# Autodesk Inventor assembly: ASY МОО 001 отстойник осветлитель
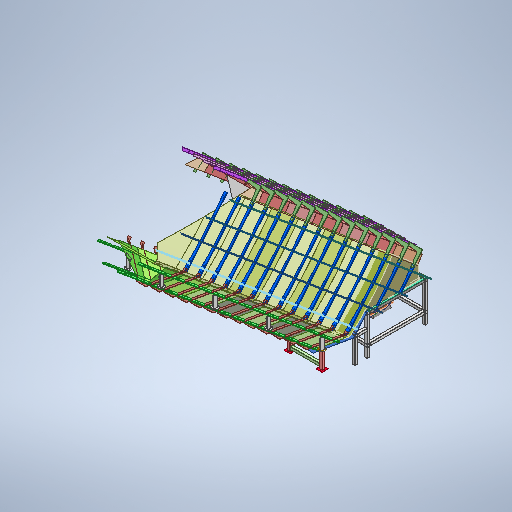
[picture p0: Inventor's stored thumbnail of the model, 512x512]
Saved by Autodesk Inventor 2025 (Build 290162010, 162A)
## iProperties
Created: 2024-04-28
Part Number: ASY МОО 001 отстойник осветлитель
Document SubType Name: Weldment
Designer: admin
Weld Material: Welded Aluminum-6061
Mass: 3.05393e+07 g
Surface Area: 3.06781e+06 cm^2
Volume: 2.84022e+07 cm^3
Density: 1.07525 g/cm^3
Author: admin
## Documents named in this file (61)
- C:\Users\admin\YandexDisk-badmisterfox\домашниий пк\Inventor\Manturovo\Manturovo_Se-clar\ASY МОО 001 отстойник осветлитель.iam
- C:\Users\admin\YandexDisk-badmisterfox\домашниий пк\Inventor\Manturovo\Manturovo_Se-clar\Пример емкости.ipt
- C:\Users\admin\YandexDisk-badmisterfox\домашниий пк\Inventor\Manturovo\Manturovo_Se-clar\Рама основания\ASY MSC 090 base frame.iam
- C:\Users\admin\YandexDisk-badmisterfox\домашниий пк\Inventor\Manturovo\Manturovo_Se-clar\ASY MSC 080 roсket.iam
- C:\Users\admin\YandexDisk-badmisterfox\домашниий пк\Inventor\Manturovo\Manturovo_Se-clar\ASY MSC 010 cone.iam
- C:\Users\admin\YandexDisk-badmisterfox\домашниий пк\Inventor\Manturovo\Manturovo_Se-clar\ракета\МОО 064 ракета труба.ipt
- C:\Users\admin\YandexDisk-badmisterfox\домашниий пк\Inventor\Manturovo\Manturovo_Se-clar\MSC 000 DIM settler-clarifier.ipt
- C:\Users\admin\YandexDisk-badmisterfox\домашниий пк\Inventor\Manturovo\Manturovo_Se-clar\MSC 031 sheet lowerback.ipt
- C:\Users\admin\YandexDisk-badmisterfox\домашниий пк\Inventor\Manturovo\Manturovo_Se-clar\MSC 021 sheet left board hip.ipt
- C:\Users\admin\YandexDisk-badmisterfox\домашниий пк\Inventor\Manturovo\Manturovo_Se-clar\MSC 022 sheet right board hip.ipt
- C:\Users\admin\YandexDisk-badmisterfox\домашниий пк\Inventor\Manturovo\Manturovo_Se-clar\конус\MSC 071 ridge 1.ipt
- C:\Users\admin\YandexDisk-badmisterfox\домашниий пк\Inventor\Manturovo\Manturovo_Se-clar\конус\MSC 073 ridge 3.ipt
- C:\Users\admin\YandexDisk-badmisterfox\домашниий пк\Inventor\Manturovo\Manturovo_Se-clar\конус\MSC 074 face 1.ipt
- C:\Users\admin\YandexDisk-badmisterfox\домашниий пк\Inventor\Manturovo\Manturovo_Se-clar\Content Center Files\en-US\ISO 5251 B 3D\ISO 5251 Bends 3D without straight ends(90 deg) DN150 11 11.ipt
- C:\Users\admin\YandexDisk-badmisterfox\домашниий пк\Inventor\Manturovo\Manturovo_Se-clar\Content Center Files\en-US\DIN EN 1092-1 01 - PN 25\DIN EN 1092-1 Plate Flange for Welding Type 01 - PN 25 150 x 168.3.ipt
- C:\Users\admin\YandexDisk-badmisterfox\домашниий пк\Inventor\Manturovo\Manturovo_Se-clar\МОО 061 труба верх 1.ipt
- C:\Users\admin\YandexDisk-badmisterfox\домашниий пк\Inventor\Manturovo\Manturovo_Se-clar\МОО 062 труба верх 2.ipt
- C:\Users\admin\YandexDisk-badmisterfox\домашниий пк\Inventor\Manturovo\Manturovo_Se-clar\МОО 063 труба верх 3.ipt
- C:\Users\admin\YandexDisk-badmisterfox\домашниий пк\Inventor\Manturovo\Manturovo_Se-clar\Part1.ipt
- C:\Users\admin\YandexDisk-badmisterfox\домашниий пк\Inventor\Manturovo\Manturovo_Se-clar\стапель\ASY стапель.iam
- C:\Users\admin\YandexDisk-badmisterfox\домашниий пк\Inventor\Manturovo\Manturovo_Se-clar\MSC 0101 sheet gills.ipt
- C:\Users\admin\YandexDisk-badmisterfox\домашниий пк\Inventor\Manturovo\Manturovo_Se-clar\MSC 068 stringer lowerback.ipt
- C:\Users\admin\YandexDisk-badmisterfox\домашниий пк\Inventor\Manturovo\Manturovo_Se-clar\конус\MSC 072 ridge 2.ipt
- C:\Users\admin\YandexDisk-badmisterfox\домашниий пк\Inventor\Manturovo\Manturovo_Se-clar\MSC 075 face 2.ipt
- C:\Users\admin\YandexDisk-badmisterfox\домашниий пк\Inventor\Manturovo\Manturovo_Se-clar\MSC 076 face 3.ipt
- C:\Users\admin\YandexDisk-badmisterfox\домашниий пк\Inventor\Manturovo\Manturovo_Se-clar\MSC 077 face 4.ipt
- C:\Users\admin\YandexDisk-badmisterfox\домашниий пк\Inventor\Manturovo\Manturovo_Se-clar\MSC 110 revision hatch 1.ipt
- C:\Users\admin\YandexDisk-badmisterfox\домашниий пк\Inventor\Manturovo\Manturovo_Se-clar\MSC 035 ring.ipt
- C:\Users\admin\YandexDisk-badmisterfox\домашниий пк\Inventor\Manturovo\Manturovo_Se-clar\MSC 074 ridge 4.ipt
- C:\Users\admin\YandexDisk-badmisterfox\домашниий пк\Inventor\Manturovo\Manturovo_Se-clar\MSC 075 ridge 5.ipt
- C:\Users\admin\YandexDisk-badmisterfox\домашниий пк\Inventor\Manturovo\Manturovo_Se-clar\MSC 081 pillar 1.ipt
- C:\Users\admin\YandexDisk-badmisterfox\домашниий пк\Inventor\Manturovo\Manturovo_Se-clar\MSC 036 flange 500.ipt
- C:\Users\admin\YandexDisk-badmisterfox\домашниий пк\Inventor\Manturovo\Manturovo_Se-clar\MSC 037 flange cover 500.ipt
- C:\Users\admin\YandexDisk-badmisterfox\домашниий пк\Inventor\Manturovo\Manturovo_Se-clar\MSC 038 flange cover ring 500.ipt
- C:\Users\admin\YandexDisk-badmisterfox\домашниий пк\Inventor\Manturovo\Manturovo_Se-clar\MSC 039 flange cover plate 500.ipt
- C:\Users\admin\YandexDisk-badmisterfox\домашниий пк\Inventor\Manturovo\Manturovo_Se-clar\Content Center Files\en-US\DIN EN ISO 8676\DIN EN ISO 8676 - M12 x 1,5 x 30.ipt
- C:\Users\admin\YandexDisk-badmisterfox\домашниий пк\Inventor\Manturovo\Manturovo_Se-clar\Content Center Files\en-US\ISO 4032(2)\ISO 4032 - M12 - ISO.ipt
- C:\Users\admin\YandexDisk-badmisterfox\домашниий пк\Inventor\Manturovo\Manturovo_Se-clar\Рама основания\ASY MSC 120  base frame.iam
- C:\Users\admin\YandexDisk-badmisterfox\домашниий пк\Inventor\Manturovo\Manturovo_Se-clar\Рама основания\ASY MSC 121  base frame.iam
- C:\Users\admin\YandexDisk-badmisterfox\домашниий пк\Inventor\Manturovo\Manturovo_Se-clar\Чертеж для парам. рамы.ipt
- C:\Users\admin\YandexDisk-badmisterfox\домашниий пк\Inventor\Manturovo\Manturovo_Se-clar\ASY MSC 120.1  base frame.iam
- C:\Users\admin\YandexDisk-badmisterfox\домашниий пк\Inventor\Manturovo\Manturovo_Se-clar\ASY MSC 122  base frame.iam
- C:\Users\admin\YandexDisk-badmisterfox\домашниий пк\Inventor\Manturovo\Manturovo_Se-clar\ASY MSC 123  base frame.iam
- C:\Users\admin\YandexDisk-badmisterfox\домашниий пк\Inventor\Manturovo\Manturovo_Se-clar\ASY MSC 124  base frame.iam
- C:\Users\admin\YandexDisk-badmisterfox\домашниий пк\Inventor\Manturovo\Manturovo_Se-clar\MSC 125 base tube.ipt
- C:\Users\admin\YandexDisk-badmisterfox\домашниий пк\Inventor\Manturovo\Manturovo_Se-clar\MSC 126 flange base tube.ipt
- C:\Users\admin\YandexDisk-badmisterfox\домашниий пк\Inventor\Manturovo\Manturovo_Se-clar\MSC 128 flange base tube support.ipt
- C:\Users\admin\YandexDisk-badmisterfox\домашниий пк\Inventor\Manturovo\Manturovo_Se-clar\MSC 125 base tube_MIR2.ipt
- C:\Users\admin\YandexDisk-badmisterfox\домашниий пк\Inventor\Manturovo\Manturovo_Se-clar\DXF файлы\MSC 126 flange base tube_MIR2.ipt
- C:\Users\admin\YandexDisk-badmisterfox\домашниий пк\Inventor\Manturovo\Manturovo_Se-clar\DXF файлы\MSC 128 flange base tube support_MIR1.ipt
- C:\Users\admin\YandexDisk-badmisterfox\домашниий пк\Inventor\Manturovo\Manturovo_Se-clar\ASY MSC 201 BACK.iam
- C:\Users\admin\YandexDisk-badmisterfox\домашниий пк\Inventor\Manturovo\Manturovo_Se-clar\ASY MSC 202 LEFT BOARD.iam
- C:\Users\admin\YandexDisk-badmisterfox\домашниий пк\Inventor\Manturovo\Manturovo_Se-clar\ASY MSC 203 RIGHT BOARD.iam
- C:\Users\admin\YandexDisk-badmisterfox\домашниий пк\Inventor\Manturovo\Manturovo_Se-clar\ASY MSC 204 BELLY.iam
- C:\Users\admin\YandexDisk-badmisterfox\домашниий пк\Inventor\Manturovo\Manturovo_Se-clar\MSC 063 stringer board #.ipt
- C:\Users\admin\YandexDisk-badmisterfox\домашниий пк\Inventor\Manturovo\Manturovo_Se-clar\MSC 064 stringer board ##.ipt
- C:\Users\admin\YandexDisk-badmisterfox\домашниий пк\Inventor\Manturovo\Manturovo_Se-clar\MSC 055 rib hip 2.ipt
- C:\Users\admin\YandexDisk-badmisterfox\домашниий пк\Inventor\Manturovo\Manturovo_Se-clar\MSC 054 rib hip 1.ipt
- C:\Users\admin\YandexDisk-badmisterfox\домашниий пк\Inventor\Manturovo\Manturovo_Se-clar\MSC 077 screen pillar .iam
- C:\Users\admin\YandexDisk-badmisterfox\домашниий пк\Inventor\Manturovo\Manturovo_Se-clar\MSC 0102 sheet gills.ipt
- C:\Users\admin\YandexDisk-badmisterfox\домашниий пк\Inventor\Manturovo\Manturovo_Se-clar\MSC 078 creen pillar.iam
## Components (131 placed, 62 different names)
1. Пример емкости.ipt:1 — Mate:1, Mate:2, Flush:2
2. MSC 000 DIM settler-clarifier.ipt:1
3. ASY MSC 090 base frame.iam:1 [sub-assembly] — Flush:19, Flush:21, Flush:82, Mate:82
4. ASY MSC 010 cone.iam:1 [sub-assembly] — Flush:22, Mate:16, Flush:28, Mate:65, Mate:78, Tangent:11, Flush:79, Mate:82, Mate:83
5. ASY MSC 080 roсket.iam:1 [sub-assembly] — Flush:23
6. МОО 064 ракета труба.ipt:1
7. MSC 031 sheet lowerback.ipt:1 — Mate:15, Mate:16, Tangent:10, Tangent:11, Tangent:12, Cylindrical:2, Rigid:185
8. MSC 021 sheet left board hip.ipt:1 — Flush:41, Mate:78
9. MSC 022 sheet right board hip.ipt:1 — Mate:30
10. MSC 071 ridge 1.ipt:1 — Mate:50, Flush:57, Mate:68, Flush:81, Flush:83, Mate:85
11. MSC 074 face 1.ipt:1 — Rigid:156, Rigid:157, Flush:62, Rigid:159, Mate:80
12. MSC 073 ridge 3.ipt:1 — Flush:57, Mate:68, Mate:77, Flush:78, Mate:81, Flush:80
13. DIN EN 1092-1 Plate Flange for Welding Type 01 - PN 25 150 x 168.3.ipt:1 — Rigid:158
14. МОО 061 труба верх 1.ipt:1 — Rigid:158, Rigid:59, Rigid:159
15. ISO 5251 Bends 3D without straight ends(90 deg) DN150 11 11.ipt:1 — Rigid:59, Rotational:2
16. МОО 062 труба верх 2.ipt:1 — Rigid:132, Rigid:156
17. DIN EN 1092-1 Plate Flange for Welding Type 01 - PN 25 150 x 168.3.ipt:2 — Rigid:132
18. МОО 063 труба верх 3.ipt:1 — Rigid:157
19. Part1.ipt:1
20. ASY стапель.iam:1 [sub-assembly] — Mate:63
21. MSC 068 stringer lowerback.ipt:1 — Mate:65, Tangent:10
22. MSC 072 ridge 2.ipt:1 — Flush:58, Mate:81, Flush:80, Flush:81, Flush:84
23. МОО 061 труба верх 1.ipt:2 — Rotational:2
24. MSC 075 face 2.ipt:1 — Flush:61, Mate:76
25. MSC 076 face 3.ipt:1 — Flush:76, Mate:76
26. MSC 077 face 4.ipt:1 — Mate:77, Flush:77, Flush:78, Mate:80
27. MSC 110 revision hatch 1:1 — Flush:82
28. MSC 068 stringer lowerback:2 — Mate:83, Tangent:12
29. MSC 035 ring:1 — Cylindrical:2, Rigid:185, Rigid:186
30. MSC 074 ridge 4:1 — Flush:83, Mate:85, Flush:84, Rigid:173
31. MSC 075 ridge 5:1 — Rigid:173
32. MSC 081 pillar 1:1 — Insert:1, Insert:2, Insert:3, Insert:4, Rigid:179
33. MSC 036 flange 500:1 — Rigid:175
34. MSC 036 flange 500:2 — Rigid:175, Rigid:176, Rigid:186
35. MSC 036 flange 500:3 — Rigid:176, Rigid:177, Mate:87
36. MSC 036 flange 500:4 — Rigid:177, Rotational:4
37. MSC 037 flange cover 500:1 — Rotational:4, Mate:87, Rigid:178, Mate:108
38. MSC 038 flange cover ring 500:1 — Rigid:178, Mate:109, Tangent:15
39. DIN EN ISO 8676 M12 x 1,5 x 30:1 — Rigid:179
40. ISO 4032 M12:1 — Insert:2
41. ISO 4032 M12:2 — Insert:1
42. ISO 4032 M12:3 — Insert:3
43. ISO 4032 M12:4 — Insert:4
44. ASY MSC 120  base frame:1 [sub-assembly] — Flush:93, Mate:97, Rotational:5
45. ASY MSC 121  base frame:1 [sub-assembly] — Mate:98, Flush:95, Mate:99
46. Чертеж для парам. рамы:1 — Flush:94, Mate:95, Mate:97, Mate:99, Mate:100, Mate:103, Mate:105, Mate:107
47. ASY MSC 120.1  base frame:2 [sub-assembly] — Flush:96, Mate:100, Mate:101
48. ASY MSC 122  base frame:2 [sub-assembly] — Flush:97, Mate:102, Mate:103
49. ASY MSC 123  base frame:2 [sub-assembly] — Flush:98, Mate:104, Mate:105
50. ASY MSC 124  base frame:2 [sub-assembly] — Flush:99, Mate:106, Mate:107
51. ASY MSC 201 BACK:1 [sub-assembly] — Mate:110
52. MSC 055 rib hip 2:2
53. MSC 063 stringer board #.ipt:2
54. MSC 064 stringer board ##.ipt:2
55. MSC 054 rib board hip 1:2
56. ASY MSC 202 LEFT BOARD:1 [sub-assembly]
57. MSC 063 stringer board #.ipt:1
58. MSC 054 rib board hip 1:1
59. MSC 055 rib hip 2:1
60. MSC 064 stringer board ##.ipt:1
61. ASY MSC 203 RIGHT BOARD:1 [sub-assembly]
62. ASY MSC 204 BELLY:1 [sub-assembly] — Mate:111
63. MSC 077 screen pillar :1 [sub-assembly] — Mate:111, Flush:100, Mate:112, Flush:101, Mate:113
64. MSC 0102 sheet gills:1 — Mate:113
65. MSC 078 creen pillar:1 [sub-assembly]
66. MSC 126 flange base tube_MIR2:1 — Rigid:183
67. MSC 125 base tube_MIR2:1 — Rigid:183, Rigid:184
68. MSC 128 flange base tube support_MIR1:1 — Rigid:184
69. MSC 125 base tube:1 — Rigid:180, Rigid:182
70. MSC 128 flange base tube support:1 — Rigid:182
71. MSC 126 flange base tube:1 — Rigid:180, Rotational:5
72. MSC 126 flange base tube_MIR2:2
73. MSC 125 base tube_MIR2:2
74. MSC 128 flange base tube support_MIR1:2
75. MSC 125 base tube:2
76. MSC 128 flange base tube support:2
77. MSC 126 flange base tube:2
78. MSC 126 flange base tube_MIR2:3
79. MSC 125 base tube_MIR2:3
80. MSC 128 flange base tube support_MIR1:3
81. MSC 125 base tube:3
82. MSC 128 flange base tube support:3
83. MSC 126 flange base tube:3
84. MSC 126 flange base tube_MIR2:4
85. MSC 125 base tube_MIR2:4
86. MSC 128 flange base tube support_MIR1:4
87. MSC 125 base tube:4
88. MSC 128 flange base tube support:4
89. MSC 126 flange base tube:4
90. MSC 039 flange cover plate 500:1 — Mate:108, Mate:109, Tangent:15
91. MSC 039 flange cover plate 500:2
92. MSC 039 flange cover plate 500:3
93. MSC 039 flange cover plate 500:4
94. MSC 039 flange cover plate 500:5
95. MSC 039 flange cover plate 500:6
96. MSC 039 flange cover plate 500:7
97. MSC 039 flange cover plate 500:8
98. MSC 039 flange cover plate 500:9
99. MSC 039 flange cover plate 500:10
100. MSC 039 flange cover plate 500:11
101. MSC 039 flange cover plate 500:12
102. MSC 0101 sheet gills.ipt:1 — Mate:112, Flush:101
103. MSC 0101 sheet gills:2
104. MSC 0101 sheet gills:3
105. MSC 0101 sheet gills:4
106. MSC 0101 sheet gills:5
107. MSC 0101 sheet gills:6
108. MSC 0101 sheet gills:7
109. MSC 0101 sheet gills:8
110. MSC 0101 sheet gills:9
111. MSC 0101 sheet gills:10
112. MSC 0101 sheet gills:11
113. MSC 0101 sheet gills:12
114. MSC 0101 sheet gills:13
115. MSC 0101 sheet gills:14
116. MSC 0101 sheet gills:15
117. MSC 0101 sheet gills:16
118. MSC 0101 sheet gills:17
119. MSC 0101 sheet gills:18
120. MSC 0101 sheet gills:19
121. MSC 0101 sheet gills:20
122. MSC 0101 sheet gills:21
123. MSC 0101 sheet gills:22
124. MSC 0101 sheet gills:23
125. MSC 0101 sheet gills:24
126. MSC 0101 sheet gills:25
127. MSC 0101 sheet gills:26
128. MSC 0101 sheet gills:27
129. MSC 0101 sheet gills:28
130. MSC 0101 sheet gills:29
131. MSC 0101 sheet gills:30
## Component patterns: (4 elements, first: MSC 126 flange base tube_MIR2:1 + MSC 125 base tube_MIR2:1 + MSC 128 flange base tube support_MIR1:1 + MSC 125 base tube:1 + MSC 128 flange base tube support:1 + MSC 126 flange base tube:1), (12 elements, first: MSC 039 flange cover plate 500:1), (30 elements, first: MSC 0101 sheet gills.ipt:1)
## Relationships (150: Mate 56, Flush 41, WeldJoint 36, Tangent 9, Insert 4, RevoluteJoint 3, CylindricalJoint 1)
- Mate:1: Пример емкости.ipt:1
- Mate:2: Пример емкости.ipt:1
- Flush:2: Пример емкости.ipt:1
- [Flush]: ASY MSC 201 BACK:1
- [Mate]: ASY MSC 204 BELLY:1
- [Flush]: ASY MSC 201 BACK:1
- Flush:19: ASY MSC 090 base frame.iam:1
- Flush:21: ASY MSC 090 base frame.iam:1
- Flush:22: ASY MSC 010 cone.iam:1
- Flush:23: ASY MSC 080 roсket.iam:1
- Mate:15: MSC 031 sheet lowerback.ipt:1
- [Flush]: ASY MSC 201 BACK:1
- Mate:16: ASY MSC 010 cone.iam:1 ↔ MSC 031 sheet lowerback.ipt:1
- Flush:28: ASY MSC 010 cone.iam:1
- [Flush]: ASY MSC 202 LEFT BOARD:1
- [Tangent]: ASY MSC 201 BACK:1 ↔ ASY MSC 202 LEFT BOARD:1
- [Mate]: ASY MSC 201 BACK:1
- Flush:41: MSC 021 sheet left board hip.ipt:1
- [Flush]: MSC 021 sheet left board hip.ipt:1 ↔ ASY MSC 201 BACK:1
- [Tangent]: MSC 021 sheet left board hip.ipt:1 ↔ ASY MSC 201 BACK:1
- Mate:30: MSC 022 sheet right board hip.ipt:1
- [Flush]: MSC 022 sheet right board hip.ipt:1 ↔ ASY MSC 201 BACK:1
- [Tangent]: MSC 022 sheet right board hip.ipt:1 ↔ ASY MSC 201 BACK:1
- [Mate]: ASY MSC 010 cone.iam:1 ↔ ASY MSC 201 BACK:1
- [Mate]: ASY MSC 010 cone.iam:1 ↔ ASY MSC 202 LEFT BOARD:1
- [Flush]: ASY MSC 202 LEFT BOARD:1
- [Tangent]: ASY MSC 201 BACK:1 ↔ ASY MSC 202 LEFT BOARD:1
- Mate:50 (200 mm): MSC 071 ridge 1.ipt:1
- [Mate]: ASY MSC 010 cone.iam:1 ↔ ASY MSC 204 BELLY:1
- [Mate]: ASY MSC 202 LEFT BOARD:1 ↔ ASY MSC 204 BELLY:1
- Rigid:158 [WeldJoint]: DIN EN 1092-1 Plate Flange for Welding Type 01 - PN 25 150 x 168.3.ipt:1 ↔ МОО 061 труба верх 1.ipt:1
- Rigid:59 [WeldJoint]: МОО 061 труба верх 1.ipt:1 ↔ ISO 5251 Bends 3D without straight ends(90 deg) DN150 11 11.ipt:1
- [Mate]: ASY MSC 010 cone.iam:1 ↔ ASY MSC 203 RIGHT BOARD:1
- [Mate]: ASY MSC 203 RIGHT BOARD:1
- [Tangent]: ASY MSC 201 BACK:1 ↔ ASY MSC 203 RIGHT BOARD:1
- [WeldJoint] (-50 mm): ASY MSC 201 BACK:1 ↔ ASY MSC 202 LEFT BOARD:1
- [WeldJoint] (-50 mm): ASY MSC 201 BACK:1 ↔ ASY MSC 203 RIGHT BOARD:1
- [Flush]: ASY MSC 202 LEFT BOARD:1 ↔ ASY MSC 204 BELLY:1
- [Mate]: ASY MSC 202 LEFT BOARD:1 ↔ ASY MSC 204 BELLY:1
- [Mate]: ASY стапель.iam:1 ↔ ASY MSC 201 BACK:1
- [Flush]: ASY стапель.iam:1 ↔ ASY MSC 201 BACK:1
- Mate:63: ASY стапель.iam:1
- Rigid:132 [WeldJoint]: МОО 062 труба верх 2.ipt:1 ↔ DIN EN 1092-1 Plate Flange for Welding Type 01 - PN 25 150 x 168.3.ipt:2
- Mate:65: ASY MSC 010 cone.iam:1 ↔ MSC 068 stringer lowerback.ipt:1
- [Mate]: MSC 068 stringer lowerback.ipt:1 ↔ ASY MSC 201 BACK:1
- Tangent:10: MSC 031 sheet lowerback.ipt:1 ↔ MSC 068 stringer lowerback.ipt:1
- [WeldJoint] (-50 mm): ASY MSC 201 BACK:1 ↔ ASY MSC 202 LEFT BOARD:1
- [WeldJoint] (-50 mm): ASY MSC 201 BACK:1 ↔ ASY MSC 203 RIGHT BOARD:1
- [Flush]: ASY MSC 202 LEFT BOARD:1 ↔ ASY MSC 204 BELLY:1
- [Mate]: ASY MSC 202 LEFT BOARD:1 ↔ ASY MSC 204 BELLY:1
- [Flush] (200 mm): MSC 073 ridge 3.ipt:1 ↔ ASY MSC 202 LEFT BOARD:1
- Flush:57: MSC 071 ridge 1.ipt:1 ↔ MSC 073 ridge 3.ipt:1
- Mate:68: MSC 071 ridge 1.ipt:1 ↔ MSC 073 ridge 3.ipt:1
- Flush:58 (200 mm): MSC 072 ridge 2.ipt:1
- Rotational:2 [RevoluteJoint]: ISO 5251 Bends 3D without straight ends(90 deg) DN150 11 11.ipt:1 ↔ МОО 061 труба верх 1.ipt:2
- [Mate]: MSC 075 face 2.ipt:1 ↔ ASY MSC 202 LEFT BOARD:1
- [Flush]: MSC 075 face 2.ipt:1 ↔ ASY MSC 202 LEFT BOARD:1
- Flush:61: MSC 075 face 2.ipt:1
- Rigid:156 [WeldJoint]: MSC 074 face 1.ipt:1 ↔ МОО 062 труба верх 2.ipt:1
- Rigid:157 [WeldJoint]: MSC 074 face 1.ipt:1 ↔ МОО 063 труба верх 3.ipt:1
- [Mate]: MSC 074 face 1.ipt:1 ↔ ASY MSC 204 BELLY:1
- Flush:62: MSC 074 face 1.ipt:1
- [Mate]: MSC 074 face 1.ipt:1 ↔ ASY MSC 204 BELLY:1
- Rigid:159 [WeldJoint] (-200 mm): MSC 074 face 1.ipt:1 ↔ МОО 061 труба верх 1.ipt:1
- Flush:76: MSC 076 face 3.ipt:1
- [Mate]: MSC 076 face 3.ipt:1 ↔ ASY MSC 202 LEFT BOARD:1
- Mate:76: MSC 075 face 2.ipt:1 ↔ MSC 076 face 3.ipt:1
- Mate:77: MSC 073 ridge 3.ipt:1 ↔ MSC 077 face 4.ipt:1
- Flush:77: MSC 077 face 4.ipt:1
- Flush:78: MSC 073 ridge 3.ipt:1 ↔ MSC 077 face 4.ipt:1
- Mate:78: ASY MSC 010 cone.iam:1 ↔ MSC 021 sheet left board hip.ipt:1
- Tangent:11 (22 mm): ASY MSC 010 cone.iam:1 ↔ MSC 031 sheet lowerback.ipt:1
- Flush:79: ASY MSC 010 cone.iam:1
- Mate:80: MSC 074 face 1.ipt:1 ↔ MSC 077 face 4.ipt:1
- Mate:81: MSC 073 ridge 3.ipt:1 ↔ MSC 072 ridge 2.ipt:1
- Flush:80: MSC 073 ridge 3.ipt:1 ↔ MSC 072 ridge 2.ipt:1
- Flush:81: MSC 071 ridge 1.ipt:1 ↔ MSC 072 ridge 2.ipt:1
- [WeldJoint] (-50 mm): ASY MSC 201 BACK:1 ↔ MSC 055 rib hip 2:2
- Flush:82: ASY MSC 090 base frame.iam:1 ↔ MSC 110 revision hatch 1:1
- Mate:82: ASY MSC 090 base frame.iam:1 ↔ ASY MSC 010 cone.iam:1
- [WeldJoint] (-50 mm): ASY MSC 201 BACK:1 ↔ MSC 054 rib board hip 1:2
- [WeldJoint] (-50 mm): ASY MSC 201 BACK:1 ↔ MSC 055 rib hip 2:1
- [WeldJoint] (-50 mm): ASY MSC 201 BACK:1 ↔ MSC 054 rib board hip 1:1
- Mate:83: ASY MSC 010 cone.iam:1 ↔ MSC 068 stringer lowerback:2
- [Mate]: MSC 068 stringer lowerback:2 ↔ ASY MSC 201 BACK:1
- Tangent:12: MSC 031 sheet lowerback.ipt:1 ↔ MSC 068 stringer lowerback:2
- Flush:83: MSC 071 ridge 1.ipt:1 ↔ MSC 074 ridge 4:1
- Mate:85: MSC 071 ridge 1.ipt:1 ↔ MSC 074 ridge 4:1
- Flush:84: MSC 072 ridge 2.ipt:1 ↔ MSC 074 ridge 4:1
- Rigid:173 [WeldJoint]: MSC 074 ridge 4:1 ↔ MSC 075 ridge 5:1
- Rigid:175 [WeldJoint]: MSC 036 flange 500:1 ↔ MSC 036 flange 500:2
- Rigid:176 [WeldJoint]: MSC 036 flange 500:2 ↔ MSC 036 flange 500:3
- Rigid:177 [WeldJoint]: MSC 036 flange 500:3 ↔ MSC 036 flange 500:4
- Cylindrical:2: MSC 031 sheet lowerback.ipt:1 ↔ MSC 035 ring:1
- Rotational:4 [RevoluteJoint]: MSC 036 flange 500:4 ↔ MSC 037 flange cover 500:1
- Mate:87: MSC 036 flange 500:3 ↔ MSC 037 flange cover 500:1
- Rigid:178 [WeldJoint]: MSC 037 flange cover 500:1 ↔ MSC 038 flange cover ring 500:1
- Insert:1: MSC 081 pillar 1:1 ↔ ISO 4032 M12:2
- Insert:2: MSC 081 pillar 1:1 ↔ ISO 4032 M12:1
- Insert:3: MSC 081 pillar 1:1 ↔ ISO 4032 M12:3
- Insert:4: MSC 081 pillar 1:1 ↔ ISO 4032 M12:4
- Rigid:179 [WeldJoint] (-3 mm): MSC 081 pillar 1:1 ↔ DIN EN ISO 8676 M12 x 1,5 x 30:1
- Flush:93 (-3 mm): ASY MSC 120  base frame:1
- [Mate]: ASY MSC 120  base frame:1
- [Mate]: MSC 081 pillar 1:1 ↔ ASY MSC 204 BELLY:1
- Flush:94: Чертеж для парам. рамы:1
- Mate:95: Чертеж для парам. рамы:1
- [Mate]: Чертеж для парам. рамы:1 ↔ ASY MSC 204 BELLY:1
- Mate:97: ASY MSC 120  base frame:1 ↔ Чертеж для парам. рамы:1
- Mate:98: ASY MSC 121  base frame:1
- Flush:95 (-3 mm): ASY MSC 121  base frame:1
- Mate:99: ASY MSC 121  base frame:1 ↔ Чертеж для парам. рамы:1
- Flush:96 (-3 mm): ASY MSC 120.1  base frame:2
- Mate:100: Чертеж для парам. рамы:1 ↔ ASY MSC 120.1  base frame:2
- Mate:101: ASY MSC 120.1  base frame:2
- Flush:97 (-3 mm): ASY MSC 122  base frame:2
- Mate:102: ASY MSC 122  base frame:2
- Mate:103: Чертеж для парам. рамы:1 ↔ ASY MSC 122  base frame:2
- Flush:98 (-3 mm): ASY MSC 123  base frame:2
- Mate:104: ASY MSC 123  base frame:2
- Mate:105: Чертеж для парам. рамы:1 ↔ ASY MSC 123  base frame:2
- Flush:99 (-3 mm): ASY MSC 124  base frame:2
- Mate:106: ASY MSC 124  base frame:2
- Mate:107: Чертеж для парам. рамы:1 ↔ ASY MSC 124  base frame:2
- Rigid:180 [WeldJoint]: MSC 125 base tube:1 ↔ MSC 126 flange base tube:1
- Rotational:5 [RevoluteJoint]: ASY MSC 120  base frame:1 ↔ MSC 126 flange base tube:1
- Rigid:182 [WeldJoint]: MSC 125 base tube:1 ↔ MSC 128 flange base tube support:1
- Rigid:183 [WeldJoint]: MSC 126 flange base tube_MIR2:1 ↔ MSC 125 base tube_MIR2:1
- Rigid:184 [WeldJoint]: MSC 125 base tube_MIR2:1 ↔ MSC 128 flange base tube support_MIR1:1
- Mate:110: ASY MSC 201 BACK:1
- Rigid:185 [WeldJoint] (20 mm): MSC 031 sheet lowerback.ipt:1 ↔ MSC 035 ring:1
- Mate:108: MSC 037 flange cover 500:1 ↔ MSC 039 flange cover plate 500:1
- Mate:109: MSC 038 flange cover ring 500:1 ↔ MSC 039 flange cover plate 500:1
- Tangent:15: MSC 038 flange cover ring 500:1 ↔ MSC 039 flange cover plate 500:1
- Rigid:186 [WeldJoint]: MSC 035 ring:1 ↔ MSC 036 flange 500:2
- [WeldJoint]: MSC 063 stringer board #.ipt:1 ↔ ASY MSC 203 RIGHT BOARD:1
- [WeldJoint]: MSC 064 stringer board ##.ipt:1 ↔ ASY MSC 203 RIGHT BOARD:1
- [WeldJoint] (2 mm): MSC 064 stringer board ##.ipt:1 ↔ ASY MSC 203 RIGHT BOARD:1
- [WeldJoint] (500 mm): MSC 055 rib hip 2:1 ↔ ASY MSC 203 RIGHT BOARD:1
- [WeldJoint] (500 mm): MSC 054 rib board hip 1:1 ↔ MSC 055 rib hip 2:1
- [WeldJoint]: MSC 063 stringer board #.ipt:2 ↔ ASY MSC 202 LEFT BOARD:1
- [WeldJoint]: MSC 064 stringer board ##.ipt:2 ↔ ASY MSC 202 LEFT BOARD:1
- [WeldJoint] (2 mm): MSC 064 stringer board ##.ipt:2 ↔ ASY MSC 202 LEFT BOARD:1
- [WeldJoint] (500 mm): MSC 055 rib hip 2:2 ↔ ASY MSC 202 LEFT BOARD:1
- [WeldJoint] (500 mm): MSC 055 rib hip 2:2 ↔ MSC 054 rib board hip 1:2
- Mate:111: ASY MSC 204 BELLY:1 ↔ MSC 077 screen pillar :1
- Flush:100: MSC 077 screen pillar :1
- Mate:112: MSC 077 screen pillar :1 ↔ MSC 0101 sheet gills.ipt:1
- Flush:101: MSC 077 screen pillar :1 ↔ MSC 0101 sheet gills.ipt:1
- Mate:113: MSC 077 screen pillar :1 ↔ MSC 0102 sheet gills:1
## Named parameters: Бак_нахлест_фланца = 25 mm, d384_d346 = 0 mm, d386_d341 = 0 mm, d388_d243 = -50 mm, d389_d246 = -50 mm, Шаг_опор_по_баку = 2000 mm
